# Autodesk Inventor assembly: PCB_PCB_N2-final launch PCB1_2022-10-12 (9) 1
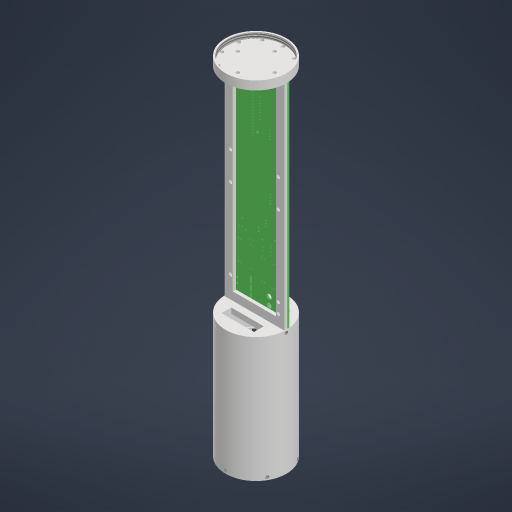
[picture p0: Inventor's stored thumbnail of the model, 512x512]
Saved by Autodesk Inventor 2023 (Build 270158000, 158)
## iProperties
Company: Kicad
Created: 2022-10-12
Part Number: PCB_PCB_N2-final launch PCB1_2022-10-12 (9) 1
Description: KiCad electronic assembly
Document SubType Name: Assembly
Designer: Mike
Authority: Unknown
Title: PCB_PCB_N2-final launch PCB1_2022-10-12 (9).step
Author: Pcbnew
Sending System: KiCad to STEP converter
Preprocessor: Open CASCADE STEP processor 7.5
## Documents named in this file (4)
- C:\Users\Mike\Downloads\PCB_PCB_N2-final launch PCB1_2022-10-12 (9).iam
- C:\Users\Mike\Downloads\_autosave-PCB_PCB_N2-final launch PCB1_2022-10-12 (9) PCB.ipt
- C:\Users\Mike\Downloads\case v0.ipt
- C:\Users\Mike\Downloads\battery holder.ipt
## Components (3 placed, 3 different names)
1. 1 — Mate:1, Mate:2
2. case v0:1 — Mate:1, Mate:2, Mate:3
3. battery holder:1 — Mate:3
## Relationships (3: Mate 3)
- Mate:1: 1 ↔ case v0:1
- Mate:2: 1 ↔ case v0:1
- Mate:3: case v0:1 ↔ battery holder:1
